# Autodesk Inventor assembly: om_HIKOROBO_2.0
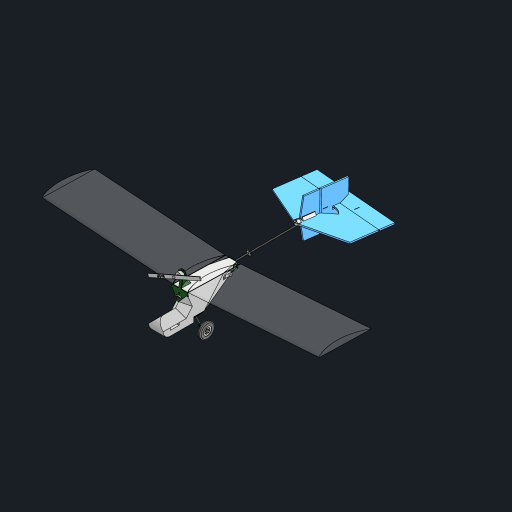
[picture p0: Inventor's stored thumbnail of the model, 512x512]
Saved by Autodesk Inventor 2023 (Build 270158000, 158)
## iProperties
Created: 2022-06-22
Part Number: om_HIKOROBO_2.0
Document SubType Name: Assembly
Designer: legot
Author: legot
## Documents named in this file (15)
- C:\Users\legot\Documents\Inventor\HIKOSAPO\OM\om_HIKOROBO_2.0.iam
- C:\Users\legot\Documents\Inventor\HIKOSAPO\OM\om_Body_2.0.ipt
- C:\Users\legot\Documents\Inventor\HIKOSAPO\OM\om_MotorMount_2.0.ipt
- C:\Users\legot\Documents\Inventor\HIKOSAPO\Drop\om_Drop.iam
- C:\Users\legot\Documents\Inventor\HIKOSAPO\public_parts\MainMotor.ipt
- C:\Users\legot\Documents\Inventor\HIKOSAPO\public_parts\Propeller.ipt
- C:\Users\legot\Documents\Inventor\HIKOSAPO\Gear\GearV1.iam
- C:\Users\legot\Documents\Inventor\HIKOSAPO\public_parts\Tail_Set.iam
- C:\Users\legot\Documents\Inventor\HIKOSAPO\public_parts\MainWing.ipt
- C:\Users\legot\Documents\Inventor\HIKOSAPO\public_parts\chicken.ipt
- C:\Users\legot\Documents\Inventor\HIKOSAPO\public_parts\MainRod.ipt
- C:\Users\legot\Documents\Inventor\HIKOSAPO\public_parts\ServoMotor.ipt
- C:\Users\legot\Documents\Inventor\HIKOSAPO\public_parts\ServoMotor_Holder.ipt
- C:\Users\legot\Documents\Inventor\HIKOSAPO\public_parts\WireHolder.ipt
- C:\Users\legot\Documents\Inventor\HIKOSAPO\OM\om_BackHolder.ipt
## Components (17 placed, 14 different names)
1. om_Body_2.0:1 — メイト:1, メイト:7, メイト:8, フラッシュ:2, メイト:10, メイト:11, フラッシュ:6, メイト:12, メイト:13, メイト:14, メイト:17, メイト:19, メイト:20, メイト:25, メイト:26, メイト:27, メイト:28, メイト:32, メイト:36, メイト:37, メイト:38
2. om_MotorMount_2.0:1 — メイト:1, メイト:7, メイト:8, 挿入:1, 挿入:2, 正接:1, メイト:21, メイト:22
3. MainMotor:1 — 挿入:1, 挿入:2, 挿入:3
4. Propeller:1 — 挿入:3
5. GearV1:1 [sub-assembly] — フラッシュ:2, メイト:10, メイト:11
6. MainWing:1 — フラッシュ:6, メイト:17, 正接:1, 正接:2, 正接:3
7. om_Drop:1 [sub-assembly] — メイト:12, メイト:13, メイト:14
8. chicken:1 — メイト:19, 正接:2
9. chicken:2 — メイト:20, 正接:3
10. MainRod:1 — メイト:21, メイト:22, メイト:39, メイト:40
11. Tail_Set:1 [sub-assembly]
12. ServoMotor:1 — メイト:27, メイト:28, メイト:33, メイト:34, メイト:35
13. ServoMotor:2 — メイト:25, メイト:26, メイト:29, メイト:30, メイト:31
14. ServoMotor_Holder:1 — メイト:33, メイト:34, メイト:35, メイト:36
15. ServoMotor_Holder:2 — メイト:29, メイト:30, メイト:31, メイト:32
16. WireHolder:1 — メイト:39, メイト:40
17. om_BackHolder:1 — メイト:37, メイト:38
## Relationships (37: Mate 29, Insert 3, Tangent 3, Flush 2)
- メイト:1 [Mate]: om_Body_2.0:1 ↔ om_MotorMount_2.0:1
- メイト:7 [Mate]: om_Body_2.0:1 ↔ om_MotorMount_2.0:1
- メイト:8 [Mate]: om_Body_2.0:1 ↔ om_MotorMount_2.0:1
- フラッシュ:2 [Flush]: om_Body_2.0:1 ↔ GearV1:1
- メイト:10 [Mate]: om_Body_2.0:1 ↔ GearV1:1
- メイト:11 [Mate]: om_Body_2.0:1 ↔ GearV1:1
- フラッシュ:6 [Flush]: om_Body_2.0:1 ↔ MainWing:1
- メイト:12 [Mate]: om_Body_2.0:1 ↔ om_Drop:1
- メイト:13 [Mate]: om_Body_2.0:1 ↔ om_Drop:1
- メイト:14 [Mate]: om_Body_2.0:1 ↔ om_Drop:1
- 挿入:1 [Insert]: om_MotorMount_2.0:1 ↔ MainMotor:1
- 挿入:2 [Insert]: om_MotorMount_2.0:1 ↔ MainMotor:1
- 挿入:3 [Insert]: MainMotor:1 ↔ Propeller:1
- メイト:17 [Mate]: om_Body_2.0:1 ↔ MainWing:1
- 正接:1 [Tangent]: om_MotorMount_2.0:1 ↔ MainWing:1
- メイト:19 [Mate]: om_Body_2.0:1 ↔ chicken:1
- 正接:2 [Tangent]: MainWing:1 ↔ chicken:1
- メイト:20 [Mate]: om_Body_2.0:1 ↔ chicken:2
- 正接:3 [Tangent]: MainWing:1 ↔ chicken:2
- メイト:21 [Mate]: om_MotorMount_2.0:1 ↔ MainRod:1
- メイト:22 [Mate]: om_MotorMount_2.0:1 ↔ MainRod:1
- メイト:25 [Mate]: om_Body_2.0:1 ↔ ServoMotor:2
- メイト:26 [Mate]: om_Body_2.0:1 ↔ ServoMotor:2
- メイト:27 [Mate]: om_Body_2.0:1 ↔ ServoMotor:1
- メイト:28 [Mate]: om_Body_2.0:1 ↔ ServoMotor:1
- メイト:29 [Mate]: ServoMotor:2 ↔ ServoMotor_Holder:2
- メイト:30 [Mate]: ServoMotor:2 ↔ ServoMotor_Holder:2
- メイト:31 [Mate]: ServoMotor:2 ↔ ServoMotor_Holder:2
- メイト:32 [Mate]: om_Body_2.0:1 ↔ ServoMotor_Holder:2
- メイト:33 [Mate]: ServoMotor:1 ↔ ServoMotor_Holder:1
- メイト:34 [Mate]: ServoMotor:1 ↔ ServoMotor_Holder:1
- メイト:35 [Mate]: ServoMotor:1 ↔ ServoMotor_Holder:1
- メイト:36 [Mate]: om_Body_2.0:1 ↔ ServoMotor_Holder:1
- メイト:37 [Mate]: om_Body_2.0:1 ↔ om_BackHolder:1
- メイト:38 [Mate]: om_Body_2.0:1 ↔ om_BackHolder:1
- メイト:39 [Mate]: MainRod:1 ↔ WireHolder:1
- メイト:40 [Mate]: MainRod:1 ↔ WireHolder:1
